# Autodesk Inventor assembly: WheelAssembly3.0
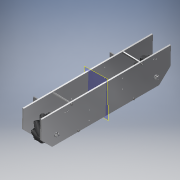
[picture p0: Inventor's stored thumbnail of the model, 180x180]
Saved by Autodesk Inventor 2019 (Build 230136000, 136)
## iProperties
Created: 2017-07-22
Part Number: WheelAssembly3.0
Document SubType Name: Assembly
Designer: User
Mass: 2301.48 g
Surface Area: 4071.67 cm^2
Volume: 902.346 cm^3
Density: 2.55055 g/cm^3
Author: User
## Documents named in this file (23)
- C:\Robotics\CAD\2020-21-CAD\Drivetrain\InvertedDriveTrain.iam
- C:\Robotics\CAD\COTSParts\Actobotics\615 parts\615398.25inBoreBeveledGears.ipt
- C:\Robotics\CAD\2016-17_CAD\Custom COTS\4inax.ipt
- C:\Robotics\CAD\COTSParts\Wheels\4in Wheel Intergreated Hub 8mm Rev2.ipt
- C:\Robotics\CAD\COTSParts\Actobotics\Thrust Bearings\6655K13.ipt
- C:\Robotics\CAD\2018-19_CAD\Offseason\InvertedDrivePlateOutside.ipt
- C:\Robotics\CAD\2018-19_CAD\Offseason\InvertedDrivePlateInside.ipt
- C:\Robotics\CAD\COTSParts\Actobotics\535 parts\535198Bearing.25ID.5OD.ipt
- C:\Robotics\CAD\COTSParts\Actobotics\Collar.ipt
- C:\Robotics\CAD\COTSParts\Fasteners\6-32 SHCS x500.ipt
- C:\Robotics\CAD\COTSParts\Fasteners\Hex Standoff 6-32 x2250.ipt
- C:\Robotics\CAD\COTSParts\Motors\am-3102NeveRest20 (1)_MIR.ipt
- C:\Robotics\CAD\COTSParts\Rev\REV-41-1657MecanumWheelRight.iam
- C:\Robotics\CAD\2020-21-CAD\Drivetrain\motor mount.ipt
- C:\Robotics\CAD\COTSParts\Tetrix\Tetrix hub - motor.ipt
- C:\Robotics\CAD\COTSParts\Actobotics\615 parts\615398.25inBoreBeveledGears_MIR1.ipt
- C:\Robotics\CAD\2016-17_CAD\Custom COTS\4inax_MIR1.ipt
- C:\Robotics\CAD\COTSParts\Actobotics\Thrust Bearings\6655K13_MIR1.ipt
- C:\Robotics\CAD\COTSParts\Actobotics\535 parts\535198Bearing.25ID.5OD_MIR1.ipt
- C:\Robotics\CAD\COTSParts\Actobotics\Collar_MIR1.ipt
- C:\Robotics\CAD\COTSParts\Rev\REV-41-1657MecanumWheelRight_MIR.iam
- C:\Robotics\CAD\2020-21-CAD\Drivetrain\motor mount_MIR.ipt
- C:\Robotics\CAD\COTSParts\Motors\am-3102NeveRest20 (1)_MIR_MIR.ipt
## Components (39 placed, 22 different names)
1. 615398.25inBoreBeveledGears:2 — Insert:47, Mate:40, Rotation:6
2. 615398.25inBoreBeveledGears:3 — Insert:77, Mate:40, Mate:45, Rotation:6
3. 4inax:4 — Insert:147, Mate:45, Mate:63, Mate:69
4. 4in Wheel Intergreated Hub 8mm Rev2:1
5. 4in Wheel Intergreated Hub 8mm Rev2:2
6. 6655K13:2 — Insert:77, Mate:44
7. 6655K13:4 — Insert:47, Mate:68
8. InvertedDrivePlateOutside:1 — Insert:71, Insert:128, Insert:129, Insert:130, Insert:131, Insert:136, Insert:137, Insert:138, Insert:139, Symmetry:1
9. InvertedDrivePlateInside:1 — Insert:90, Insert:132, Insert:133, Insert:134, Insert:135, Insert:140, Insert:141, Insert:142, Insert:143, Mate:44, Symmetry:1, Mate:65, Flush:10, Flush:11, Angle:1, Mate:73
10. 535198Bearing.25ID.5OD:1 — Insert:71, Insert:86
11. Collar:1 — Insert:86, Insert:147
12. 535198Bearing.25ID.5OD:5 — Insert:90
13. Hex Standoff 6-32 x2250:1 — Insert:129, Insert:134
14. Hex Standoff 6-32 x2250:2 — Insert:128, Insert:132
15. Hex Standoff 6-32 x2250:3 — Insert:131, Insert:135
16. Hex Standoff 6-32 x2250:4 — Insert:130, Insert:133
17. 6-32 SHCS x500:22 — Insert:136
18. 6-32 SHCS x500:23 — Insert:137
19. 6-32 SHCS x500:24 — Insert:138
20. 6-32 SHCS x500:25 — Insert:139
21. 6-32 SHCS x500:26 — Insert:140
22. 6-32 SHCS x500:27 — Insert:141
23. 6-32 SHCS x500:28 — Insert:142
24. 6-32 SHCS x500:29 — Insert:143
25. REV-41-1657MecanumWheelRight:1 [sub-assembly] — Mate:63, Mate:70, Mate:71, Mate:72
26. motor mount:1 — Mate:65, Flush:10, Mate:66, Mate:67, Flush:11
27. am-3102NeveRest20 (1)_MIR:2 — Mate:66, Mate:67, Mate:68, Angle:1
28. Tetrix hub - motor:1 — Mate:69, Mate:70, Mate:71, Mate:72, Mate:73
29. 615398.25inBoreBeveledGears_MIR1:1 — Rotation:7, Mate:74, Insert:149
30. 615398.25inBoreBeveledGears_MIR1:2 — Rotation:7, Mate:74, Mate:75, Insert:148
31. 4inax_MIR1:1 — Mate:75, Insert:150, Mate:76
32. 6655K13_MIR1:1 — Insert:148
33. 6655K13_MIR1:2 — Insert:149, Mate:77
34. 535198Bearing.25ID.5OD_MIR1:1 — Insert:151
35. Collar_MIR1:1 — Insert:150, Insert:151
36. 535198Bearing.25ID.5OD_MIR1:2
37. REV-41-1657MecanumWheelRight_MIR:1 [sub-assembly] — Mate:76
38. motor mount_MIR:1 — Mate:78, Mate:79
39. am-3102NeveRest20 (1)_MIR_MIR:1 — Mate:77, Mate:78, Mate:79
## Relationships (51: Insert 26, Mate 19, RelateRotation 2, Flush 2, Symmetry 1, Angle 1)
- Insert:47: 615398.25inBoreBeveledGears:2 ↔ 6655K13:4
- Insert:71: InvertedDrivePlateOutside:1 ↔ 535198Bearing.25ID.5OD:1
- Insert:77: 615398.25inBoreBeveledGears:3 ↔ 6655K13:2
- Insert:86: 535198Bearing.25ID.5OD:1 ↔ Collar:1
- Insert:90: InvertedDrivePlateInside:1 ↔ 535198Bearing.25ID.5OD:5
- Insert:128: InvertedDrivePlateOutside:1 ↔ Hex Standoff 6-32 x2250:2
- Insert:129: InvertedDrivePlateOutside:1 ↔ Hex Standoff 6-32 x2250:1
- Insert:130: InvertedDrivePlateOutside:1 ↔ Hex Standoff 6-32 x2250:4
- Insert:131: InvertedDrivePlateOutside:1 ↔ Hex Standoff 6-32 x2250:3
- Insert:132: InvertedDrivePlateInside:1 ↔ Hex Standoff 6-32 x2250:2
- Insert:133: InvertedDrivePlateInside:1 ↔ Hex Standoff 6-32 x2250:4
- Insert:134: InvertedDrivePlateInside:1 ↔ Hex Standoff 6-32 x2250:1
- Insert:135: InvertedDrivePlateInside:1 ↔ Hex Standoff 6-32 x2250:3
- Insert:136: InvertedDrivePlateOutside:1 ↔ 6-32 SHCS x500:22
- Insert:137: InvertedDrivePlateOutside:1 ↔ 6-32 SHCS x500:23
- Insert:138: InvertedDrivePlateOutside:1 ↔ 6-32 SHCS x500:24
- Insert:139: InvertedDrivePlateOutside:1 ↔ 6-32 SHCS x500:25
- Insert:140: InvertedDrivePlateInside:1 ↔ 6-32 SHCS x500:26
- Insert:141: InvertedDrivePlateInside:1 ↔ 6-32 SHCS x500:27
- Insert:142: InvertedDrivePlateInside:1 ↔ 6-32 SHCS x500:28
- Insert:143: InvertedDrivePlateInside:1 ↔ 6-32 SHCS x500:29
- Insert:147: 4inax:4 ↔ Collar:1
- Mate:40 (-7.6197 mm): 615398.25inBoreBeveledGears:2 ↔ 615398.25inBoreBeveledGears:3
- Mate:44: 6655K13:2 ↔ InvertedDrivePlateInside:1
- Mate:45: 615398.25inBoreBeveledGears:3 ↔ 4inax:4
- Rotation:6 [RelateRotation] (1 ul): 615398.25inBoreBeveledGears:2 ↔ 615398.25inBoreBeveledGears:3
- Symmetry:1: InvertedDrivePlateOutside:1 ↔ InvertedDrivePlateInside:1
- Mate:63: 4inax:4 ↔ REV-41-1657MecanumWheelRight:1
- Mate:65: InvertedDrivePlateInside:1 ↔ motor mount:1
- Flush:10 (88.9 mm): InvertedDrivePlateInside:1 ↔ motor mount:1
- Mate:66: motor mount:1 ↔ am-3102NeveRest20 (1)_MIR:2
- Mate:67: motor mount:1 ↔ am-3102NeveRest20 (1)_MIR:2
- Mate:68: 6655K13:4 ↔ am-3102NeveRest20 (1)_MIR:2
- Flush:11 (-12.7 mm): InvertedDrivePlateInside:1 ↔ motor mount:1
- Angle:1 (11.35 deg): InvertedDrivePlateInside:1 ↔ am-3102NeveRest20 (1)_MIR:2
- Mate:69: 4inax:4 ↔ Tetrix hub - motor:1
- Mate:70: REV-41-1657MecanumWheelRight:1 ↔ Tetrix hub - motor:1
- Mate:71: REV-41-1657MecanumWheelRight:1 ↔ Tetrix hub - motor:1
- Mate:72: REV-41-1657MecanumWheelRight:1 ↔ Tetrix hub - motor:1
- Mate:73 (19.05 mm): InvertedDrivePlateInside:1 ↔ Tetrix hub - motor:1
- Rotation:7 [RelateRotation] (1 ul): 615398.25inBoreBeveledGears_MIR1:1 ↔ 615398.25inBoreBeveledGears_MIR1:2
- Mate:74 (-7.6197 mm): 615398.25inBoreBeveledGears_MIR1:1 ↔ 615398.25inBoreBeveledGears_MIR1:2
- Mate:75: 615398.25inBoreBeveledGears_MIR1:2 ↔ 4inax_MIR1:1
- Insert:148: 615398.25inBoreBeveledGears_MIR1:2 ↔ 6655K13_MIR1:1
- Insert:149: 615398.25inBoreBeveledGears_MIR1:1 ↔ 6655K13_MIR1:2
- Insert:150: 4inax_MIR1:1 ↔ Collar_MIR1:1
- Insert:151: 535198Bearing.25ID.5OD_MIR1:1 ↔ Collar_MIR1:1
- Mate:76: 4inax_MIR1:1 ↔ REV-41-1657MecanumWheelRight_MIR:1
- Mate:77: 6655K13_MIR1:2 ↔ am-3102NeveRest20 (1)_MIR_MIR:1
- Mate:78: motor mount_MIR:1 ↔ am-3102NeveRest20 (1)_MIR_MIR:1
- Mate:79: motor mount_MIR:1 ↔ am-3102NeveRest20 (1)_MIR_MIR:1
